# Autodesk Inventor assembly: SAR320
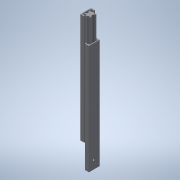
[picture p0: Inventor's stored thumbnail of the model, 180x180]
Saved by Autodesk Inventor 2020 (Build 240168000, 168)
## iProperties
Created: 2020-01-12
Part Number: SAR320
Catalog Web Link: www.cadenas.de
Description: SAR3-Slide Rails - Aluminum Alloy - Three-Step Slide Rails
Vendor: MISUMI
Document SubType Name: Assembly
Designer: psadmin
Manufacturer: MISUMI
Category: PARTsolutions
Company: MISUMI
PSOL_IDENT_0: {$CADENAS_DATA\23d-libs\misumi\metric\07_slide_rails\sar3_asmtab.prj},168 {VTYP=3D},{STYP=ASSTAB},{N
PSOL_IDENT_1: B=SAR320},{LINA=SAR320},{NN=SAR3},{DATE=09.09.2019 15:26:52},{GEOMDATE=01.03.2017 00:48:28},{VERSION=
PSOL_IDENT_2: },{LINEID=10},{WBVAR=NO},{WBNUMERIC=NO}  {NB=SAR320},{LINA=SAR320},{KT=DUMMY},{PN=SAR320},{TP=SAR3},
PSOL_IDENT_3: {TYPE=SAR3},{MAT1=Aluminum Alloy},{ST1=Clear Anodizing},{MAT2=Aluminum Alloy},{ST2=Clear Anodizing},
PSOL_IDENT_4: {MAT3=Steel},{NO=20},{RL=200},{TD=223},{A=85},{B=170},{C=85},{D=170},{RLO=147},{PPATH=sar3_series\\s
PSOL_IDENT_5: ar3_templ.prj}
NN: SAR3
NT: Slide Rails - Aluminum Alloy - Three-Step Slide Rails
NB: SAR320
NBSYN: $PN.
LINA: SAR320
PN: SAR320
TP: SAR3
MAT1: Aluminum Alloy
ST1: Clear Anodizing
MAT2: Aluminum Alloy
ST2: Clear Anodizing
MAT3: Steel
NO: 20
RL: 200
TD: 223
A: 85
B: 170
C: 85
D: 170
RLO: 147
SUPPLIER: MISUMI
ARTICLENO: SAR320
BOMINFO: SAR320
CREATOR: CADENAS GmbH
Title: SAR320
Author: Cadenas PARTsolutions
Comments: Slide Rails - Aluminum Alloy - Three-Step Slide Rails
## Documents named in this file (4)
- C:\Users\tdmp4\OneDrive\Documents\GitHub\CAD-2020\Misumi\SAR320.iam
- C:\Users\tdmp4\Downloads\SAR320_Autodesk_Inventor_2018_20200112\AIS2018\SAR320-20_r.ipt
- C:\Users\tdmp4\Downloads\SAR320_Autodesk_Inventor_2018_20200112\AIS2018\SAR320-20_b.ipt
- C:\Users\tdmp4\Downloads\SAR320_Autodesk_Inventor_2018_20200112\AIS2018\SAR3_ba.ipt
## Components (71 placed, 3 different names)
1. SAR320-20_r:1 — to_body_Z@1 <-> to_rail_Z@2, to_body_YZ@1 <-> to_rail_YZ@2, to_body2_Z@1 <-> to_rail_Z@3, to_body2_YZ@1 <-> to_rail_YZ@3, to_ball1_1_XY@1 <-> to_rail_XY@4, to_ball1_1_Z@1 <-> to_rail_Z@4, to_ball1_1_YZ@1 <-> to_rail_YZ@4, to_ball1_2_XY@1 <-> to_rail_XY@5, to_ball1_2_Z@1 <-> to_rail_Z@5, to_ball1_2_YZ@1 <-> to_rail_YZ@5, to_ball1_3_XY@1 <-> to_rail_XY@6, to_ball1_3_Z@1 <-> to_rail_Z@6, to_ball1_3_YZ@1 <-> to_rail_YZ@6, to_ball1_4_XY@1 <-> to_rail_XY@7, to_ball1_4_Z@1 <-> to_rail_Z@7, to_ball1_4_YZ@1 <-> to_rail_YZ@7, to_ball1_5_XY@1 <-> to_rail_XY@8, to_ball1_5_Z@1 <-> to_rail_Z@8, to_ball1_5_YZ@1 <-> to_rail_YZ@8, to_ball1_6_XY@1 <-> to_rail_XY@9, to_ball1_6_Z@1 <-> to_rail_Z@9, to_ball1_6_YZ@1 <-> to_rail_YZ@9, to_ball1_7_XY@1 <-> to_rail_XY@10, to_ball1_7_Z@1 <-> to_rail_Z@10, to_ball1_7_YZ@1 <-> to_rail_YZ@10, to_ball1_8_XY@1 <-> to_rail_XY@11, to_ball1_8_Z@1 <-> to_rail_Z@11, to_ball1_8_YZ@1 <-> to_rail_YZ@11, to_ball1_9_XY@1 <-> to_rail_XY@12, to_ball1_9_Z@1 <-> to_rail_Z@12, to_ball1_9_YZ@1 <-> to_rail_YZ@12, to_ball1_10_XY@1 <-> to_rail_XY@13, to_ball1_10_Z@1 <-> to_rail_Z@13, to_ball1_10_YZ@1 <-> to_rail_YZ@13, to_ball1_11_XY@1 <-> to_rail_XY@14, to_ball1_11_Z@1 <-> to_rail_Z@14, to_ball1_11_YZ@1 <-> to_rail_YZ@14, to_ball1_12_XY@1 <-> to_rail_XY@15, to_ball1_12_Z@1 <-> to_rail_Z@15, to_ball1_12_YZ@1 <-> to_rail_YZ@15, to_ball1_13_XY@1 <-> to_rail_XY@16, to_ball1_13_Z@1 <-> to_rail_Z@16, to_ball1_13_YZ@1 <-> to_rail_YZ@16, to_ball1_14_XY@1 <-> to_rail_XY@17, to_ball1_14_Z@1 <-> to_rail_Z@17, to_ball1_14_YZ@1 <-> to_rail_YZ@17, to_ball1_15_XY@1 <-> to_rail_XY@18, to_ball1_15_Z@1 <-> to_rail_Z@18, to_ball1_15_YZ@1 <-> to_rail_YZ@18, to_ball1_16_XY@1 <-> to_rail_XY@19, to_ball1_16_Z@1 <-> to_rail_Z@19, to_ball1_16_YZ@1 <-> to_rail_YZ@19, to_ball1_17_XY@1 <-> to_rail_XY@20, to_ball1_17_Z@1 <-> to_rail_Z@20, to_ball1_17_YZ@1 <-> to_rail_YZ@20, to_ball2_1_XY@1 <-> to_rail_XY@21, to_ball2_1_Z@1 <-> to_rail_Z@21, to_ball2_1_YZ@1 <-> to_rail_YZ@21, to_ball2_2_XY@1 <-> to_rail_XY@22, to_ball2_2_Z@1 <-> to_rail_Z@22, to_ball2_2_YZ@1 <-> to_rail_YZ@22, to_ball2_3_XY@1 <-> to_rail_XY@23, to_ball2_3_Z@1 <-> to_rail_Z@23, to_ball2_3_YZ@1 <-> to_rail_YZ@23, to_ball2_4_XY@1 <-> to_rail_XY@24, to_ball2_4_Z@1 <-> to_rail_Z@24, to_ball2_4_YZ@1 <-> to_rail_YZ@24, to_ball2_5_XY@1 <-> to_rail_XY@25, to_ball2_5_Z@1 <-> to_rail_Z@25, to_ball2_5_YZ@1 <-> to_rail_YZ@25, to_ball2_6_XY@1 <-> to_rail_XY@26, to_ball2_6_Z@1 <-> to_rail_Z@26, to_ball2_6_YZ@1 <-> to_rail_YZ@26, to_ball2_7_XY@1 <-> to_rail_XY@27, to_ball2_7_Z@1 <-> to_rail_Z@27, to_ball2_7_YZ@1 <-> to_rail_YZ@27, to_ball2_8_XY@1 <-> to_rail_XY@28, to_ball2_8_Z@1 <-> to_rail_Z@28, to_ball2_8_YZ@1 <-> to_rail_YZ@28, to_ball2_9_XY@1 <-> to_rail_XY@29, to_ball2_9_Z@1 <-> to_rail_Z@29, to_ball2_9_YZ@1 <-> to_rail_YZ@29, to_ball2_10_XY@1 <-> to_rail_XY@30, to_ball2_10_Z@1 <-> to_rail_Z@30, to_ball2_10_YZ@1 <-> to_rail_YZ@30, to_ball2_11_XY@1 <-> to_rail_XY@31, to_ball2_11_Z@1 <-> to_rail_Z@31, to_ball2_11_YZ@1 <-> to_rail_YZ@31, to_ball2_12_XY@1 <-> to_rail_XY@32, to_ball2_12_Z@1 <-> to_rail_Z@32, to_ball2_12_YZ@1 <-> to_rail_YZ@32, to_ball2_13_XY@1 <-> to_rail_XY@33, to_ball2_13_Z@1 <-> to_rail_Z@33, to_ball2_13_YZ@1 <-> to_rail_YZ@33, to_ball2_14_XY@1 <-> to_rail_XY@34, to_ball2_14_Z@1 <-> to_rail_Z@34, to_ball2_14_YZ@1 <-> to_rail_YZ@34, to_ball2_15_XY@1 <-> to_rail_XY@35, to_ball2_15_Z@1 <-> to_rail_Z@35, to_ball2_15_YZ@1 <-> to_rail_YZ@35, to_ball2_16_XY@1 <-> to_rail_XY@36, to_ball2_16_Z@1 <-> to_rail_Z@36, to_ball2_16_YZ@1 <-> to_rail_YZ@36, to_ball2_17_XY@1 <-> to_rail_XY@37, to_ball2_17_Z@1 <-> to_rail_Z@37, to_ball2_17_YZ@1 <-> to_rail_YZ@37, to_ball3_1_XY@1 <-> to_rail_XY@38, to_ball3_1_Z@1 <-> to_rail_Z@38, to_ball3_1_YZ@1 <-> to_rail_YZ@38, to_ball3_2_XY@1 <-> to_rail_XY@39, to_ball3_2_Z@1 <-> to_rail_Z@39, to_ball3_2_YZ@1 <-> to_rail_YZ@39, to_ball3_3_XY@1 <-> to_rail_XY@40, to_ball3_3_Z@1 <-> to_rail_Z@40, to_ball3_3_YZ@1 <-> to_rail_YZ@40, to_ball3_4_XY@1 <-> to_rail_XY@41, to_ball3_4_Z@1 <-> to_rail_Z@41, to_ball3_4_YZ@1 <-> to_rail_YZ@41, to_ball3_5_XY@1 <-> to_rail_XY@42, to_ball3_5_Z@1 <-> to_rail_Z@42, to_ball3_5_YZ@1 <-> to_rail_YZ@42, to_ball3_6_XY@1 <-> to_rail_XY@43, to_ball3_6_Z@1 <-> to_rail_Z@43, to_ball3_6_YZ@1 <-> to_rail_YZ@43, to_ball3_7_XY@1 <-> to_rail_XY@44, to_ball3_7_Z@1 <-> to_rail_Z@44, to_ball3_7_YZ@1 <-> to_rail_YZ@44, to_ball3_8_XY@1 <-> to_rail_XY@45, to_ball3_8_Z@1 <-> to_rail_Z@45, to_ball3_8_YZ@1 <-> to_rail_YZ@45, to_ball3_9_XY@1 <-> to_rail_XY@46, to_ball3_9_Z@1 <-> to_rail_Z@46, to_ball3_9_YZ@1 <-> to_rail_YZ@46, to_ball3_10_XY@1 <-> to_rail_XY@47, to_ball3_10_Z@1 <-> to_rail_Z@47, to_ball3_10_YZ@1 <-> to_rail_YZ@47, to_ball3_11_XY@1 <-> to_rail_XY@48, to_ball3_11_Z@1 <-> to_rail_Z@48, to_ball3_11_YZ@1 <-> to_rail_YZ@48, to_ball3_12_XY@1 <-> to_rail_XY@49, to_ball3_12_Z@1 <-> to_rail_Z@49, to_ball3_12_YZ@1 <-> to_rail_YZ@49, to_ball3_13_XY@1 <-> to_rail_XY@50, to_ball3_13_Z@1 <-> to_rail_Z@50, to_ball3_13_YZ@1 <-> to_rail_YZ@50, to_ball3_14_XY@1 <-> to_rail_XY@51, to_ball3_14_Z@1 <-> to_rail_Z@51, to_ball3_14_YZ@1 <-> to_rail_YZ@51, to_ball3_15_XY@1 <-> to_rail_XY@52, to_ball3_15_Z@1 <-> to_rail_Z@52, to_ball3_15_YZ@1 <-> to_rail_YZ@52, to_ball3_16_XY@1 <-> to_rail_XY@53, to_ball3_16_Z@1 <-> to_rail_Z@53, to_ball3_16_YZ@1 <-> to_rail_YZ@53, to_ball3_17_XY@1 <-> to_rail_XY@54, to_ball3_17_Z@1 <-> to_rail_Z@54, to_ball3_17_YZ@1 <-> to_rail_YZ@54, to_ball4_1_XY@1 <-> to_rail_XY@55, to_ball4_1_Z@1 <-> to_rail_Z@55, to_ball4_1_YZ@1 <-> to_rail_YZ@55, to_ball4_2_XY@1 <-> to_rail_XY@56, to_ball4_2_Z@1 <-> to_rail_Z@56, to_ball4_2_YZ@1 <-> to_rail_YZ@56, to_ball4_3_XY@1 <-> to_rail_XY@57, to_ball4_3_Z@1 <-> to_rail_Z@57, to_ball4_3_YZ@1 <-> to_rail_YZ@57, to_ball4_4_XY@1 <-> to_rail_XY@58, to_ball4_4_Z@1 <-> to_rail_Z@58, to_ball4_4_YZ@1 <-> to_rail_YZ@58, to_ball4_5_XY@1 <-> to_rail_XY@59, to_ball4_5_Z@1 <-> to_rail_Z@59, to_ball4_5_YZ@1 <-> to_rail_YZ@59, to_ball4_6_XY@1 <-> to_rail_XY@60, to_ball4_6_Z@1 <-> to_rail_Z@60, to_ball4_6_YZ@1 <-> to_rail_YZ@60, to_ball4_7_XY@1 <-> to_rail_XY@61, to_ball4_7_Z@1 <-> to_rail_Z@61, to_ball4_7_YZ@1 <-> to_rail_YZ@61, to_ball4_8_XY@1 <-> to_rail_XY@62, to_ball4_8_Z@1 <-> to_rail_Z@62, to_ball4_8_YZ@1 <-> to_rail_YZ@62, to_ball4_9_XY@1 <-> to_rail_XY@63, to_ball4_9_Z@1 <-> to_rail_Z@63, to_ball4_9_YZ@1 <-> to_rail_YZ@63, to_ball4_10_XY@1 <-> to_rail_XY@64, to_ball4_10_Z@1 <-> to_rail_Z@64, to_ball4_10_YZ@1 <-> to_rail_YZ@64, to_ball4_11_XY@1 <-> to_rail_XY@65, to_ball4_11_Z@1 <-> to_rail_Z@65, to_ball4_11_YZ@1 <-> to_rail_YZ@65, to_ball4_12_XY@1 <-> to_rail_XY@66, to_ball4_12_Z@1 <-> to_rail_Z@66, to_ball4_12_YZ@1 <-> to_rail_YZ@66, to_ball4_13_XY@1 <-> to_rail_XY@67, to_ball4_13_Z@1 <-> to_rail_Z@67, to_ball4_13_YZ@1 <-> to_rail_YZ@67, to_ball4_14_XY@1 <-> to_rail_XY@68, to_ball4_14_Z@1 <-> to_rail_Z@68, to_ball4_14_YZ@1 <-> to_rail_YZ@68, to_ball4_15_XY@1 <-> to_rail_XY@69, to_ball4_15_Z@1 <-> to_rail_Z@69, to_ball4_15_YZ@1 <-> to_rail_YZ@69, to_ball4_16_XY@1 <-> to_rail_XY@70, to_ball4_16_Z@1 <-> to_rail_Z@70, to_ball4_16_YZ@1 <-> to_rail_YZ@70, to_ball4_17_XY@1 <-> to_rail_XY@71, to_ball4_17_Z@1 <-> to_rail_Z@71, to_ball4_17_YZ@1 <-> to_rail_YZ@71
2. SAR320-20_b:1 — to_body_Z@1 <-> to_rail_Z@2, to_body_YZ@1 <-> to_rail_YZ@2
3. SAR320-20_b:2 — to_body2_Z@1 <-> to_rail_Z@3, to_body2_YZ@1 <-> to_rail_YZ@3
4. SAR3_ba:1 — to_ball1_1_XY@1 <-> to_rail_XY@4, to_ball1_1_Z@1 <-> to_rail_Z@4, to_ball1_1_YZ@1 <-> to_rail_YZ@4
5. SAR3_ba:2 — to_ball1_2_XY@1 <-> to_rail_XY@5, to_ball1_2_Z@1 <-> to_rail_Z@5, to_ball1_2_YZ@1 <-> to_rail_YZ@5
6. SAR3_ba:3 — to_ball1_3_XY@1 <-> to_rail_XY@6, to_ball1_3_Z@1 <-> to_rail_Z@6, to_ball1_3_YZ@1 <-> to_rail_YZ@6
7. SAR3_ba:4 — to_ball1_4_XY@1 <-> to_rail_XY@7, to_ball1_4_Z@1 <-> to_rail_Z@7, to_ball1_4_YZ@1 <-> to_rail_YZ@7
8. SAR3_ba:5 — to_ball1_5_XY@1 <-> to_rail_XY@8, to_ball1_5_Z@1 <-> to_rail_Z@8, to_ball1_5_YZ@1 <-> to_rail_YZ@8
9. SAR3_ba:6 — to_ball1_6_XY@1 <-> to_rail_XY@9, to_ball1_6_Z@1 <-> to_rail_Z@9, to_ball1_6_YZ@1 <-> to_rail_YZ@9
10. SAR3_ba:7 — to_ball1_7_XY@1 <-> to_rail_XY@10, to_ball1_7_Z@1 <-> to_rail_Z@10, to_ball1_7_YZ@1 <-> to_rail_YZ@10
11. SAR3_ba:8 — to_ball1_8_XY@1 <-> to_rail_XY@11, to_ball1_8_Z@1 <-> to_rail_Z@11, to_ball1_8_YZ@1 <-> to_rail_YZ@11
12. SAR3_ba:9 — to_ball1_9_XY@1 <-> to_rail_XY@12, to_ball1_9_Z@1 <-> to_rail_Z@12, to_ball1_9_YZ@1 <-> to_rail_YZ@12
13. SAR3_ba:10 — to_ball1_10_XY@1 <-> to_rail_XY@13, to_ball1_10_Z@1 <-> to_rail_Z@13, to_ball1_10_YZ@1 <-> to_rail_YZ@13
14. SAR3_ba:11 — to_ball1_11_XY@1 <-> to_rail_XY@14, to_ball1_11_Z@1 <-> to_rail_Z@14, to_ball1_11_YZ@1 <-> to_rail_YZ@14
15. SAR3_ba:12 — to_ball1_12_XY@1 <-> to_rail_XY@15, to_ball1_12_Z@1 <-> to_rail_Z@15, to_ball1_12_YZ@1 <-> to_rail_YZ@15
16. SAR3_ba:13 — to_ball1_13_XY@1 <-> to_rail_XY@16, to_ball1_13_Z@1 <-> to_rail_Z@16, to_ball1_13_YZ@1 <-> to_rail_YZ@16
17. SAR3_ba:14 — to_ball1_14_XY@1 <-> to_rail_XY@17, to_ball1_14_Z@1 <-> to_rail_Z@17, to_ball1_14_YZ@1 <-> to_rail_YZ@17
18. SAR3_ba:15 — to_ball1_15_XY@1 <-> to_rail_XY@18, to_ball1_15_Z@1 <-> to_rail_Z@18, to_ball1_15_YZ@1 <-> to_rail_YZ@18
19. SAR3_ba:16 — to_ball1_16_XY@1 <-> to_rail_XY@19, to_ball1_16_Z@1 <-> to_rail_Z@19, to_ball1_16_YZ@1 <-> to_rail_YZ@19
20. SAR3_ba:17 — to_ball1_17_XY@1 <-> to_rail_XY@20, to_ball1_17_Z@1 <-> to_rail_Z@20, to_ball1_17_YZ@1 <-> to_rail_YZ@20
21. SAR3_ba:18 — to_ball2_1_XY@1 <-> to_rail_XY@21, to_ball2_1_Z@1 <-> to_rail_Z@21, to_ball2_1_YZ@1 <-> to_rail_YZ@21
22. SAR3_ba:19 — to_ball2_2_XY@1 <-> to_rail_XY@22, to_ball2_2_Z@1 <-> to_rail_Z@22, to_ball2_2_YZ@1 <-> to_rail_YZ@22
23. SAR3_ba:20 — to_ball2_3_XY@1 <-> to_rail_XY@23, to_ball2_3_Z@1 <-> to_rail_Z@23, to_ball2_3_YZ@1 <-> to_rail_YZ@23
24. SAR3_ba:21 — to_ball2_4_XY@1 <-> to_rail_XY@24, to_ball2_4_Z@1 <-> to_rail_Z@24, to_ball2_4_YZ@1 <-> to_rail_YZ@24
25. SAR3_ba:22 — to_ball2_5_XY@1 <-> to_rail_XY@25, to_ball2_5_Z@1 <-> to_rail_Z@25, to_ball2_5_YZ@1 <-> to_rail_YZ@25
26. SAR3_ba:23 — to_ball2_6_XY@1 <-> to_rail_XY@26, to_ball2_6_Z@1 <-> to_rail_Z@26, to_ball2_6_YZ@1 <-> to_rail_YZ@26
27. SAR3_ba:24 — to_ball2_7_XY@1 <-> to_rail_XY@27, to_ball2_7_Z@1 <-> to_rail_Z@27, to_ball2_7_YZ@1 <-> to_rail_YZ@27
28. SAR3_ba:25 — to_ball2_8_XY@1 <-> to_rail_XY@28, to_ball2_8_Z@1 <-> to_rail_Z@28, to_ball2_8_YZ@1 <-> to_rail_YZ@28
29. SAR3_ba:26 — to_ball2_9_XY@1 <-> to_rail_XY@29, to_ball2_9_Z@1 <-> to_rail_Z@29, to_ball2_9_YZ@1 <-> to_rail_YZ@29
30. SAR3_ba:27 — to_ball2_10_XY@1 <-> to_rail_XY@30, to_ball2_10_Z@1 <-> to_rail_Z@30, to_ball2_10_YZ@1 <-> to_rail_YZ@30
31. SAR3_ba:28 — to_ball2_11_XY@1 <-> to_rail_XY@31, to_ball2_11_Z@1 <-> to_rail_Z@31, to_ball2_11_YZ@1 <-> to_rail_YZ@31
32. SAR3_ba:29 — to_ball2_12_XY@1 <-> to_rail_XY@32, to_ball2_12_Z@1 <-> to_rail_Z@32, to_ball2_12_YZ@1 <-> to_rail_YZ@32
33. SAR3_ba:30 — to_ball2_13_XY@1 <-> to_rail_XY@33, to_ball2_13_Z@1 <-> to_rail_Z@33, to_ball2_13_YZ@1 <-> to_rail_YZ@33
34. SAR3_ba:31 — to_ball2_14_XY@1 <-> to_rail_XY@34, to_ball2_14_Z@1 <-> to_rail_Z@34, to_ball2_14_YZ@1 <-> to_rail_YZ@34
35. SAR3_ba:32 — to_ball2_15_XY@1 <-> to_rail_XY@35, to_ball2_15_Z@1 <-> to_rail_Z@35, to_ball2_15_YZ@1 <-> to_rail_YZ@35
36. SAR3_ba:33 — to_ball2_16_XY@1 <-> to_rail_XY@36, to_ball2_16_Z@1 <-> to_rail_Z@36, to_ball2_16_YZ@1 <-> to_rail_YZ@36
37. SAR3_ba:34 — to_ball2_17_XY@1 <-> to_rail_XY@37, to_ball2_17_Z@1 <-> to_rail_Z@37, to_ball2_17_YZ@1 <-> to_rail_YZ@37
38. SAR3_ba:35 — to_ball3_1_XY@1 <-> to_rail_XY@38, to_ball3_1_Z@1 <-> to_rail_Z@38, to_ball3_1_YZ@1 <-> to_rail_YZ@38
39. SAR3_ba:36 — to_ball3_2_XY@1 <-> to_rail_XY@39, to_ball3_2_Z@1 <-> to_rail_Z@39, to_ball3_2_YZ@1 <-> to_rail_YZ@39
40. SAR3_ba:37 — to_ball3_3_XY@1 <-> to_rail_XY@40, to_ball3_3_Z@1 <-> to_rail_Z@40, to_ball3_3_YZ@1 <-> to_rail_YZ@40
41. SAR3_ba:38 — to_ball3_4_XY@1 <-> to_rail_XY@41, to_ball3_4_Z@1 <-> to_rail_Z@41, to_ball3_4_YZ@1 <-> to_rail_YZ@41
42. SAR3_ba:39 — to_ball3_5_XY@1 <-> to_rail_XY@42, to_ball3_5_Z@1 <-> to_rail_Z@42, to_ball3_5_YZ@1 <-> to_rail_YZ@42
43. SAR3_ba:40 — to_ball3_6_XY@1 <-> to_rail_XY@43, to_ball3_6_Z@1 <-> to_rail_Z@43, to_ball3_6_YZ@1 <-> to_rail_YZ@43
44. SAR3_ba:41 — to_ball3_7_XY@1 <-> to_rail_XY@44, to_ball3_7_Z@1 <-> to_rail_Z@44, to_ball3_7_YZ@1 <-> to_rail_YZ@44
45. SAR3_ba:42 — to_ball3_8_XY@1 <-> to_rail_XY@45, to_ball3_8_Z@1 <-> to_rail_Z@45, to_ball3_8_YZ@1 <-> to_rail_YZ@45
46. SAR3_ba:43 — to_ball3_9_XY@1 <-> to_rail_XY@46, to_ball3_9_Z@1 <-> to_rail_Z@46, to_ball3_9_YZ@1 <-> to_rail_YZ@46
47. SAR3_ba:44 — to_ball3_10_XY@1 <-> to_rail_XY@47, to_ball3_10_Z@1 <-> to_rail_Z@47, to_ball3_10_YZ@1 <-> to_rail_YZ@47
48. SAR3_ba:45 — to_ball3_11_XY@1 <-> to_rail_XY@48, to_ball3_11_Z@1 <-> to_rail_Z@48, to_ball3_11_YZ@1 <-> to_rail_YZ@48
49. SAR3_ba:46 — to_ball3_12_XY@1 <-> to_rail_XY@49, to_ball3_12_Z@1 <-> to_rail_Z@49, to_ball3_12_YZ@1 <-> to_rail_YZ@49
50. SAR3_ba:47 — to_ball3_13_XY@1 <-> to_rail_XY@50, to_ball3_13_Z@1 <-> to_rail_Z@50, to_ball3_13_YZ@1 <-> to_rail_YZ@50
51. SAR3_ba:48 — to_ball3_14_XY@1 <-> to_rail_XY@51, to_ball3_14_Z@1 <-> to_rail_Z@51, to_ball3_14_YZ@1 <-> to_rail_YZ@51
52. SAR3_ba:49 — to_ball3_15_XY@1 <-> to_rail_XY@52, to_ball3_15_Z@1 <-> to_rail_Z@52, to_ball3_15_YZ@1 <-> to_rail_YZ@52
53. SAR3_ba:50 — to_ball3_16_XY@1 <-> to_rail_XY@53, to_ball3_16_Z@1 <-> to_rail_Z@53, to_ball3_16_YZ@1 <-> to_rail_YZ@53
54. SAR3_ba:51 — to_ball3_17_XY@1 <-> to_rail_XY@54, to_ball3_17_Z@1 <-> to_rail_Z@54, to_ball3_17_YZ@1 <-> to_rail_YZ@54
55. SAR3_ba:52 — to_ball4_1_XY@1 <-> to_rail_XY@55, to_ball4_1_Z@1 <-> to_rail_Z@55, to_ball4_1_YZ@1 <-> to_rail_YZ@55
56. SAR3_ba:53 — to_ball4_2_XY@1 <-> to_rail_XY@56, to_ball4_2_Z@1 <-> to_rail_Z@56, to_ball4_2_YZ@1 <-> to_rail_YZ@56
57. SAR3_ba:54 — to_ball4_3_XY@1 <-> to_rail_XY@57, to_ball4_3_Z@1 <-> to_rail_Z@57, to_ball4_3_YZ@1 <-> to_rail_YZ@57
58. SAR3_ba:55 — to_ball4_4_XY@1 <-> to_rail_XY@58, to_ball4_4_Z@1 <-> to_rail_Z@58, to_ball4_4_YZ@1 <-> to_rail_YZ@58
59. SAR3_ba:56 — to_ball4_5_XY@1 <-> to_rail_XY@59, to_ball4_5_Z@1 <-> to_rail_Z@59, to_ball4_5_YZ@1 <-> to_rail_YZ@59
60. SAR3_ba:57 — to_ball4_6_XY@1 <-> to_rail_XY@60, to_ball4_6_Z@1 <-> to_rail_Z@60, to_ball4_6_YZ@1 <-> to_rail_YZ@60
61. SAR3_ba:58 — to_ball4_7_XY@1 <-> to_rail_XY@61, to_ball4_7_Z@1 <-> to_rail_Z@61, to_ball4_7_YZ@1 <-> to_rail_YZ@61
62. SAR3_ba:59 — to_ball4_8_XY@1 <-> to_rail_XY@62, to_ball4_8_Z@1 <-> to_rail_Z@62, to_ball4_8_YZ@1 <-> to_rail_YZ@62
63. SAR3_ba:60 — to_ball4_9_XY@1 <-> to_rail_XY@63, to_ball4_9_Z@1 <-> to_rail_Z@63, to_ball4_9_YZ@1 <-> to_rail_YZ@63
64. SAR3_ba:61 — to_ball4_10_XY@1 <-> to_rail_XY@64, to_ball4_10_Z@1 <-> to_rail_Z@64, to_ball4_10_YZ@1 <-> to_rail_YZ@64
65. SAR3_ba:62 — to_ball4_11_XY@1 <-> to_rail_XY@65, to_ball4_11_Z@1 <-> to_rail_Z@65, to_ball4_11_YZ@1 <-> to_rail_YZ@65
66. SAR3_ba:63 — to_ball4_12_XY@1 <-> to_rail_XY@66, to_ball4_12_Z@1 <-> to_rail_Z@66, to_ball4_12_YZ@1 <-> to_rail_YZ@66
67. SAR3_ba:64 — to_ball4_13_XY@1 <-> to_rail_XY@67, to_ball4_13_Z@1 <-> to_rail_Z@67, to_ball4_13_YZ@1 <-> to_rail_YZ@67
68. SAR3_ba:65 — to_ball4_14_XY@1 <-> to_rail_XY@68, to_ball4_14_Z@1 <-> to_rail_Z@68, to_ball4_14_YZ@1 <-> to_rail_YZ@68
69. SAR3_ba:66 — to_ball4_15_XY@1 <-> to_rail_XY@69, to_ball4_15_Z@1 <-> to_rail_Z@69, to_ball4_15_YZ@1 <-> to_rail_YZ@69
70. SAR3_ba:67 — to_ball4_16_XY@1 <-> to_rail_XY@70, to_ball4_16_Z@1 <-> to_rail_Z@70, to_ball4_16_YZ@1 <-> to_rail_YZ@70
71. SAR3_ba:68 — to_ball4_17_XY@1 <-> to_rail_XY@71, to_ball4_17_Z@1 <-> to_rail_Z@71, to_ball4_17_YZ@1 <-> to_rail_YZ@71
## Relationships (208: Mate 138, Angle 70)
- to_body_Z@1 <-> to_rail_Z@2 [Mate]: SAR320-20_r:1 ↔ SAR320-20_b:1
- to_body_YZ@1 <-> to_rail_YZ@2 [Angle] (0 deg): SAR320-20_r:1 ↔ SAR320-20_b:1
- to_body2_Z@1 <-> to_rail_Z@3 [Mate]: SAR320-20_r:1 ↔ SAR320-20_b:2
- to_body2_YZ@1 <-> to_rail_YZ@3 [Angle] (180 deg): SAR320-20_r:1 ↔ SAR320-20_b:2
- to_ball1_1_XY@1 <-> to_rail_XY@4 [Mate]: SAR320-20_r:1 ↔ SAR3_ba:1
- to_ball1_1_Z@1 <-> to_rail_Z@4 [Mate]: SAR320-20_r:1 ↔ SAR3_ba:1
- to_ball1_1_YZ@1 <-> to_rail_YZ@4 [Angle] (0 deg): SAR320-20_r:1 ↔ SAR3_ba:1
- to_ball1_2_XY@1 <-> to_rail_XY@5 [Mate]: SAR320-20_r:1 ↔ SAR3_ba:2
- to_ball1_2_Z@1 <-> to_rail_Z@5 [Mate]: SAR320-20_r:1 ↔ SAR3_ba:2
- to_ball1_2_YZ@1 <-> to_rail_YZ@5 [Angle] (0 deg): SAR320-20_r:1 ↔ SAR3_ba:2
- to_ball1_3_XY@1 <-> to_rail_XY@6 [Mate]: SAR320-20_r:1 ↔ SAR3_ba:3
- to_ball1_3_Z@1 <-> to_rail_Z@6 [Mate]: SAR320-20_r:1 ↔ SAR3_ba:3
- to_ball1_3_YZ@1 <-> to_rail_YZ@6 [Angle] (0 deg): SAR320-20_r:1 ↔ SAR3_ba:3
- to_ball1_4_XY@1 <-> to_rail_XY@7 [Mate]: SAR320-20_r:1 ↔ SAR3_ba:4
- to_ball1_4_Z@1 <-> to_rail_Z@7 [Mate]: SAR320-20_r:1 ↔ SAR3_ba:4
- to_ball1_4_YZ@1 <-> to_rail_YZ@7 [Angle] (0 deg): SAR320-20_r:1 ↔ SAR3_ba:4
- to_ball1_5_XY@1 <-> to_rail_XY@8 [Mate]: SAR320-20_r:1 ↔ SAR3_ba:5
- to_ball1_5_Z@1 <-> to_rail_Z@8 [Mate]: SAR320-20_r:1 ↔ SAR3_ba:5
- to_ball1_5_YZ@1 <-> to_rail_YZ@8 [Angle] (0 deg): SAR320-20_r:1 ↔ SAR3_ba:5
- to_ball1_6_XY@1 <-> to_rail_XY@9 [Mate]: SAR320-20_r:1 ↔ SAR3_ba:6
- to_ball1_6_Z@1 <-> to_rail_Z@9 [Mate]: SAR320-20_r:1 ↔ SAR3_ba:6
- to_ball1_6_YZ@1 <-> to_rail_YZ@9 [Angle] (0 deg): SAR320-20_r:1 ↔ SAR3_ba:6
- to_ball1_7_XY@1 <-> to_rail_XY@10 [Mate]: SAR320-20_r:1 ↔ SAR3_ba:7
- to_ball1_7_Z@1 <-> to_rail_Z@10 [Mate]: SAR320-20_r:1 ↔ SAR3_ba:7
- to_ball1_7_YZ@1 <-> to_rail_YZ@10 [Angle] (0 deg): SAR320-20_r:1 ↔ SAR3_ba:7
- to_ball1_8_XY@1 <-> to_rail_XY@11 [Mate]: SAR320-20_r:1 ↔ SAR3_ba:8
- to_ball1_8_Z@1 <-> to_rail_Z@11 [Mate]: SAR320-20_r:1 ↔ SAR3_ba:8
- to_ball1_8_YZ@1 <-> to_rail_YZ@11 [Angle] (0 deg): SAR320-20_r:1 ↔ SAR3_ba:8
- to_ball1_9_XY@1 <-> to_rail_XY@12 [Mate]: SAR320-20_r:1 ↔ SAR3_ba:9
- to_ball1_9_Z@1 <-> to_rail_Z@12 [Mate]: SAR320-20_r:1 ↔ SAR3_ba:9
- to_ball1_9_YZ@1 <-> to_rail_YZ@12 [Angle] (0 deg): SAR320-20_r:1 ↔ SAR3_ba:9
- to_ball1_10_XY@1 <-> to_rail_XY@13 [Mate]: SAR320-20_r:1 ↔ SAR3_ba:10
- to_ball1_10_Z@1 <-> to_rail_Z@13 [Mate]: SAR320-20_r:1 ↔ SAR3_ba:10
- to_ball1_10_YZ@1 <-> to_rail_YZ@13 [Angle] (0 deg): SAR320-20_r:1 ↔ SAR3_ba:10
- to_ball1_11_XY@1 <-> to_rail_XY@14 [Mate]: SAR320-20_r:1 ↔ SAR3_ba:11
- to_ball1_11_Z@1 <-> to_rail_Z@14 [Mate]: SAR320-20_r:1 ↔ SAR3_ba:11
- to_ball1_11_YZ@1 <-> to_rail_YZ@14 [Angle] (0 deg): SAR320-20_r:1 ↔ SAR3_ba:11
- to_ball1_12_XY@1 <-> to_rail_XY@15 [Mate]: SAR320-20_r:1 ↔ SAR3_ba:12
- to_ball1_12_Z@1 <-> to_rail_Z@15 [Mate]: SAR320-20_r:1 ↔ SAR3_ba:12
- to_ball1_12_YZ@1 <-> to_rail_YZ@15 [Angle] (0 deg): SAR320-20_r:1 ↔ SAR3_ba:12
- to_ball1_13_XY@1 <-> to_rail_XY@16 [Mate]: SAR320-20_r:1 ↔ SAR3_ba:13
- to_ball1_13_Z@1 <-> to_rail_Z@16 [Mate]: SAR320-20_r:1 ↔ SAR3_ba:13
- to_ball1_13_YZ@1 <-> to_rail_YZ@16 [Angle] (0 deg): SAR320-20_r:1 ↔ SAR3_ba:13
- to_ball1_14_XY@1 <-> to_rail_XY@17 [Mate]: SAR320-20_r:1 ↔ SAR3_ba:14
- to_ball1_14_Z@1 <-> to_rail_Z@17 [Mate]: SAR320-20_r:1 ↔ SAR3_ba:14
- to_ball1_14_YZ@1 <-> to_rail_YZ@17 [Angle] (0 deg): SAR320-20_r:1 ↔ SAR3_ba:14
- to_ball1_15_XY@1 <-> to_rail_XY@18 [Mate]: SAR320-20_r:1 ↔ SAR3_ba:15
- to_ball1_15_Z@1 <-> to_rail_Z@18 [Mate]: SAR320-20_r:1 ↔ SAR3_ba:15
- to_ball1_15_YZ@1 <-> to_rail_YZ@18 [Angle] (0 deg): SAR320-20_r:1 ↔ SAR3_ba:15
- to_ball1_16_XY@1 <-> to_rail_XY@19 [Mate]: SAR320-20_r:1 ↔ SAR3_ba:16
- to_ball1_16_Z@1 <-> to_rail_Z@19 [Mate]: SAR320-20_r:1 ↔ SAR3_ba:16
- to_ball1_16_YZ@1 <-> to_rail_YZ@19 [Angle] (0 deg): SAR320-20_r:1 ↔ SAR3_ba:16
- to_ball1_17_XY@1 <-> to_rail_XY@20 [Mate]: SAR320-20_r:1 ↔ SAR3_ba:17
- to_ball1_17_Z@1 <-> to_rail_Z@20 [Mate]: SAR320-20_r:1 ↔ SAR3_ba:17
- to_ball1_17_YZ@1 <-> to_rail_YZ@20 [Angle] (0 deg): SAR320-20_r:1 ↔ SAR3_ba:17
- to_ball2_1_XY@1 <-> to_rail_XY@21 [Mate]: SAR320-20_r:1 ↔ SAR3_ba:18
- to_ball2_1_Z@1 <-> to_rail_Z@21 [Mate]: SAR320-20_r:1 ↔ SAR3_ba:18
- to_ball2_1_YZ@1 <-> to_rail_YZ@21 [Angle] (0 deg): SAR320-20_r:1 ↔ SAR3_ba:18
- to_ball2_2_XY@1 <-> to_rail_XY@22 [Mate]: SAR320-20_r:1 ↔ SAR3_ba:19
- to_ball2_2_Z@1 <-> to_rail_Z@22 [Mate]: SAR320-20_r:1 ↔ SAR3_ba:19
- to_ball2_2_YZ@1 <-> to_rail_YZ@22 [Angle] (0 deg): SAR320-20_r:1 ↔ SAR3_ba:19
- to_ball2_3_XY@1 <-> to_rail_XY@23 [Mate]: SAR320-20_r:1 ↔ SAR3_ba:20
- to_ball2_3_Z@1 <-> to_rail_Z@23 [Mate]: SAR320-20_r:1 ↔ SAR3_ba:20
- to_ball2_3_YZ@1 <-> to_rail_YZ@23 [Angle] (0 deg): SAR320-20_r:1 ↔ SAR3_ba:20
- to_ball2_4_XY@1 <-> to_rail_XY@24 [Mate]: SAR320-20_r:1 ↔ SAR3_ba:21
- to_ball2_4_Z@1 <-> to_rail_Z@24 [Mate]: SAR320-20_r:1 ↔ SAR3_ba:21
- to_ball2_4_YZ@1 <-> to_rail_YZ@24 [Angle] (0 deg): SAR320-20_r:1 ↔ SAR3_ba:21
- to_ball2_5_XY@1 <-> to_rail_XY@25 [Mate]: SAR320-20_r:1 ↔ SAR3_ba:22
- to_ball2_5_Z@1 <-> to_rail_Z@25 [Mate]: SAR320-20_r:1 ↔ SAR3_ba:22
- to_ball2_5_YZ@1 <-> to_rail_YZ@25 [Angle] (0 deg): SAR320-20_r:1 ↔ SAR3_ba:22
- to_ball2_6_XY@1 <-> to_rail_XY@26 [Mate]: SAR320-20_r:1 ↔ SAR3_ba:23
- to_ball2_6_Z@1 <-> to_rail_Z@26 [Mate]: SAR320-20_r:1 ↔ SAR3_ba:23
- to_ball2_6_YZ@1 <-> to_rail_YZ@26 [Angle] (0 deg): SAR320-20_r:1 ↔ SAR3_ba:23
- to_ball2_7_XY@1 <-> to_rail_XY@27 [Mate]: SAR320-20_r:1 ↔ SAR3_ba:24
- to_ball2_7_Z@1 <-> to_rail_Z@27 [Mate]: SAR320-20_r:1 ↔ SAR3_ba:24
- to_ball2_7_YZ@1 <-> to_rail_YZ@27 [Angle] (0 deg): SAR320-20_r:1 ↔ SAR3_ba:24
- to_ball2_8_XY@1 <-> to_rail_XY@28 [Mate]: SAR320-20_r:1 ↔ SAR3_ba:25
- to_ball2_8_Z@1 <-> to_rail_Z@28 [Mate]: SAR320-20_r:1 ↔ SAR3_ba:25
- to_ball2_8_YZ@1 <-> to_rail_YZ@28 [Angle] (0 deg): SAR320-20_r:1 ↔ SAR3_ba:25
- to_ball2_9_XY@1 <-> to_rail_XY@29 [Mate]: SAR320-20_r:1 ↔ SAR3_ba:26
- to_ball2_9_Z@1 <-> to_rail_Z@29 [Mate]: SAR320-20_r:1 ↔ SAR3_ba:26
- to_ball2_9_YZ@1 <-> to_rail_YZ@29 [Angle] (0 deg): SAR320-20_r:1 ↔ SAR3_ba:26
- to_ball2_10_XY@1 <-> to_rail_XY@30 [Mate]: SAR320-20_r:1 ↔ SAR3_ba:27
- to_ball2_10_Z@1 <-> to_rail_Z@30 [Mate]: SAR320-20_r:1 ↔ SAR3_ba:27
- to_ball2_10_YZ@1 <-> to_rail_YZ@30 [Angle] (0 deg): SAR320-20_r:1 ↔ SAR3_ba:27
- to_ball2_11_XY@1 <-> to_rail_XY@31 [Mate]: SAR320-20_r:1 ↔ SAR3_ba:28
- to_ball2_11_Z@1 <-> to_rail_Z@31 [Mate]: SAR320-20_r:1 ↔ SAR3_ba:28
- to_ball2_11_YZ@1 <-> to_rail_YZ@31 [Angle] (0 deg): SAR320-20_r:1 ↔ SAR3_ba:28
- to_ball2_12_XY@1 <-> to_rail_XY@32 [Mate]: SAR320-20_r:1 ↔ SAR3_ba:29
- to_ball2_12_Z@1 <-> to_rail_Z@32 [Mate]: SAR320-20_r:1 ↔ SAR3_ba:29
- to_ball2_12_YZ@1 <-> to_rail_YZ@32 [Angle] (0 deg): SAR320-20_r:1 ↔ SAR3_ba:29
- to_ball2_13_XY@1 <-> to_rail_XY@33 [Mate]: SAR320-20_r:1 ↔ SAR3_ba:30
- to_ball2_13_Z@1 <-> to_rail_Z@33 [Mate]: SAR320-20_r:1 ↔ SAR3_ba:30
- to_ball2_13_YZ@1 <-> to_rail_YZ@33 [Angle] (0 deg): SAR320-20_r:1 ↔ SAR3_ba:30
- to_ball2_14_XY@1 <-> to_rail_XY@34 [Mate]: SAR320-20_r:1 ↔ SAR3_ba:31
- to_ball2_14_Z@1 <-> to_rail_Z@34 [Mate]: SAR320-20_r:1 ↔ SAR3_ba:31
- to_ball2_14_YZ@1 <-> to_rail_YZ@34 [Angle] (0 deg): SAR320-20_r:1 ↔ SAR3_ba:31
- to_ball2_15_XY@1 <-> to_rail_XY@35 [Mate]: SAR320-20_r:1 ↔ SAR3_ba:32
- to_ball2_15_Z@1 <-> to_rail_Z@35 [Mate]: SAR320-20_r:1 ↔ SAR3_ba:32
- to_ball2_15_YZ@1 <-> to_rail_YZ@35 [Angle] (0 deg): SAR320-20_r:1 ↔ SAR3_ba:32
- to_ball2_16_XY@1 <-> to_rail_XY@36 [Mate]: SAR320-20_r:1 ↔ SAR3_ba:33
- to_ball2_16_Z@1 <-> to_rail_Z@36 [Mate]: SAR320-20_r:1 ↔ SAR3_ba:33
- to_ball2_16_YZ@1 <-> to_rail_YZ@36 [Angle] (0 deg): SAR320-20_r:1 ↔ SAR3_ba:33
- to_ball2_17_XY@1 <-> to_rail_XY@37 [Mate]: SAR320-20_r:1 ↔ SAR3_ba:34
- to_ball2_17_Z@1 <-> to_rail_Z@37 [Mate]: SAR320-20_r:1 ↔ SAR3_ba:34
- to_ball2_17_YZ@1 <-> to_rail_YZ@37 [Angle] (0 deg): SAR320-20_r:1 ↔ SAR3_ba:34
- to_ball3_1_XY@1 <-> to_rail_XY@38 [Mate]: SAR320-20_r:1 ↔ SAR3_ba:35
- to_ball3_1_Z@1 <-> to_rail_Z@38 [Mate]: SAR320-20_r:1 ↔ SAR3_ba:35
- to_ball3_1_YZ@1 <-> to_rail_YZ@38 [Angle] (0 deg): SAR320-20_r:1 ↔ SAR3_ba:35
- to_ball3_2_XY@1 <-> to_rail_XY@39 [Mate]: SAR320-20_r:1 ↔ SAR3_ba:36
- to_ball3_2_Z@1 <-> to_rail_Z@39 [Mate]: SAR320-20_r:1 ↔ SAR3_ba:36
- to_ball3_2_YZ@1 <-> to_rail_YZ@39 [Angle] (0 deg): SAR320-20_r:1 ↔ SAR3_ba:36
- to_ball3_3_XY@1 <-> to_rail_XY@40 [Mate]: SAR320-20_r:1 ↔ SAR3_ba:37
- to_ball3_3_Z@1 <-> to_rail_Z@40 [Mate]: SAR320-20_r:1 ↔ SAR3_ba:37
- to_ball3_3_YZ@1 <-> to_rail_YZ@40 [Angle] (0 deg): SAR320-20_r:1 ↔ SAR3_ba:37
- to_ball3_4_XY@1 <-> to_rail_XY@41 [Mate]: SAR320-20_r:1 ↔ SAR3_ba:38
- to_ball3_4_Z@1 <-> to_rail_Z@41 [Mate]: SAR320-20_r:1 ↔ SAR3_ba:38
- to_ball3_4_YZ@1 <-> to_rail_YZ@41 [Angle] (0 deg): SAR320-20_r:1 ↔ SAR3_ba:38
- to_ball3_5_XY@1 <-> to_rail_XY@42 [Mate]: SAR320-20_r:1 ↔ SAR3_ba:39
- to_ball3_5_Z@1 <-> to_rail_Z@42 [Mate]: SAR320-20_r:1 ↔ SAR3_ba:39
- to_ball3_5_YZ@1 <-> to_rail_YZ@42 [Angle] (0 deg): SAR320-20_r:1 ↔ SAR3_ba:39
- to_ball3_6_XY@1 <-> to_rail_XY@43 [Mate]: SAR320-20_r:1 ↔ SAR3_ba:40
- to_ball3_6_Z@1 <-> to_rail_Z@43 [Mate]: SAR320-20_r:1 ↔ SAR3_ba:40
- to_ball3_6_YZ@1 <-> to_rail_YZ@43 [Angle] (0 deg): SAR320-20_r:1 ↔ SAR3_ba:40
- to_ball3_7_XY@1 <-> to_rail_XY@44 [Mate]: SAR320-20_r:1 ↔ SAR3_ba:41
- to_ball3_7_Z@1 <-> to_rail_Z@44 [Mate]: SAR320-20_r:1 ↔ SAR3_ba:41
- to_ball3_7_YZ@1 <-> to_rail_YZ@44 [Angle] (0 deg): SAR320-20_r:1 ↔ SAR3_ba:41
- to_ball3_8_XY@1 <-> to_rail_XY@45 [Mate]: SAR320-20_r:1 ↔ SAR3_ba:42
- to_ball3_8_Z@1 <-> to_rail_Z@45 [Mate]: SAR320-20_r:1 ↔ SAR3_ba:42
- to_ball3_8_YZ@1 <-> to_rail_YZ@45 [Angle] (0 deg): SAR320-20_r:1 ↔ SAR3_ba:42
- to_ball3_9_XY@1 <-> to_rail_XY@46 [Mate]: SAR320-20_r:1 ↔ SAR3_ba:43
- to_ball3_9_Z@1 <-> to_rail_Z@46 [Mate]: SAR320-20_r:1 ↔ SAR3_ba:43
- to_ball3_9_YZ@1 <-> to_rail_YZ@46 [Angle] (0 deg): SAR320-20_r:1 ↔ SAR3_ba:43
- to_ball3_10_XY@1 <-> to_rail_XY@47 [Mate]: SAR320-20_r:1 ↔ SAR3_ba:44
- to_ball3_10_Z@1 <-> to_rail_Z@47 [Mate]: SAR320-20_r:1 ↔ SAR3_ba:44
- to_ball3_10_YZ@1 <-> to_rail_YZ@47 [Angle] (0 deg): SAR320-20_r:1 ↔ SAR3_ba:44
- to_ball3_11_XY@1 <-> to_rail_XY@48 [Mate]: SAR320-20_r:1 ↔ SAR3_ba:45
- to_ball3_11_Z@1 <-> to_rail_Z@48 [Mate]: SAR320-20_r:1 ↔ SAR3_ba:45
- to_ball3_11_YZ@1 <-> to_rail_YZ@48 [Angle] (0 deg): SAR320-20_r:1 ↔ SAR3_ba:45
- to_ball3_12_XY@1 <-> to_rail_XY@49 [Mate]: SAR320-20_r:1 ↔ SAR3_ba:46
- to_ball3_12_Z@1 <-> to_rail_Z@49 [Mate]: SAR320-20_r:1 ↔ SAR3_ba:46
- to_ball3_12_YZ@1 <-> to_rail_YZ@49 [Angle] (0 deg): SAR320-20_r:1 ↔ SAR3_ba:46
- to_ball3_13_XY@1 <-> to_rail_XY@50 [Mate]: SAR320-20_r:1 ↔ SAR3_ba:47
- to_ball3_13_Z@1 <-> to_rail_Z@50 [Mate]: SAR320-20_r:1 ↔ SAR3_ba:47
- to_ball3_13_YZ@1 <-> to_rail_YZ@50 [Angle] (0 deg): SAR320-20_r:1 ↔ SAR3_ba:47
- to_ball3_14_XY@1 <-> to_rail_XY@51 [Mate]: SAR320-20_r:1 ↔ SAR3_ba:48
- to_ball3_14_Z@1 <-> to_rail_Z@51 [Mate]: SAR320-20_r:1 ↔ SAR3_ba:48
- to_ball3_14_YZ@1 <-> to_rail_YZ@51 [Angle] (0 deg): SAR320-20_r:1 ↔ SAR3_ba:48
- to_ball3_15_XY@1 <-> to_rail_XY@52 [Mate]: SAR320-20_r:1 ↔ SAR3_ba:49
- to_ball3_15_Z@1 <-> to_rail_Z@52 [Mate]: SAR320-20_r:1 ↔ SAR3_ba:49
- to_ball3_15_YZ@1 <-> to_rail_YZ@52 [Angle] (0 deg): SAR320-20_r:1 ↔ SAR3_ba:49
- to_ball3_16_XY@1 <-> to_rail_XY@53 [Mate]: SAR320-20_r:1 ↔ SAR3_ba:50
- to_ball3_16_Z@1 <-> to_rail_Z@53 [Mate]: SAR320-20_r:1 ↔ SAR3_ba:50
- to_ball3_16_YZ@1 <-> to_rail_YZ@53 [Angle] (0 deg): SAR320-20_r:1 ↔ SAR3_ba:50
- to_ball3_17_XY@1 <-> to_rail_XY@54 [Mate]: SAR320-20_r:1 ↔ SAR3_ba:51
- to_ball3_17_Z@1 <-> to_rail_Z@54 [Mate]: SAR320-20_r:1 ↔ SAR3_ba:51
- to_ball3_17_YZ@1 <-> to_rail_YZ@54 [Angle] (0 deg): SAR320-20_r:1 ↔ SAR3_ba:51
- to_ball4_1_XY@1 <-> to_rail_XY@55 [Mate]: SAR320-20_r:1 ↔ SAR3_ba:52
- to_ball4_1_Z@1 <-> to_rail_Z@55 [Mate]: SAR320-20_r:1 ↔ SAR3_ba:52
- to_ball4_1_YZ@1 <-> to_rail_YZ@55 [Angle] (0 deg): SAR320-20_r:1 ↔ SAR3_ba:52
- to_ball4_2_XY@1 <-> to_rail_XY@56 [Mate]: SAR320-20_r:1 ↔ SAR3_ba:53
- to_ball4_2_Z@1 <-> to_rail_Z@56 [Mate]: SAR320-20_r:1 ↔ SAR3_ba:53
- to_ball4_2_YZ@1 <-> to_rail_YZ@56 [Angle] (0 deg): SAR320-20_r:1 ↔ SAR3_ba:53
- to_ball4_3_XY@1 <-> to_rail_XY@57 [Mate]: SAR320-20_r:1 ↔ SAR3_ba:54
- to_ball4_3_Z@1 <-> to_rail_Z@57 [Mate]: SAR320-20_r:1 ↔ SAR3_ba:54
- to_ball4_3_YZ@1 <-> to_rail_YZ@57 [Angle] (0 deg): SAR320-20_r:1 ↔ SAR3_ba:54
- to_ball4_4_XY@1 <-> to_rail_XY@58 [Mate]: SAR320-20_r:1 ↔ SAR3_ba:55
- to_ball4_4_Z@1 <-> to_rail_Z@58 [Mate]: SAR320-20_r:1 ↔ SAR3_ba:55
- to_ball4_4_YZ@1 <-> to_rail_YZ@58 [Angle] (0 deg): SAR320-20_r:1 ↔ SAR3_ba:55
- to_ball4_5_XY@1 <-> to_rail_XY@59 [Mate]: SAR320-20_r:1 ↔ SAR3_ba:56
- to_ball4_5_Z@1 <-> to_rail_Z@59 [Mate]: SAR320-20_r:1 ↔ SAR3_ba:56
- to_ball4_5_YZ@1 <-> to_rail_YZ@59 [Angle] (0 deg): SAR320-20_r:1 ↔ SAR3_ba:56
- to_ball4_6_XY@1 <-> to_rail_XY@60 [Mate]: SAR320-20_r:1 ↔ SAR3_ba:57
- to_ball4_6_Z@1 <-> to_rail_Z@60 [Mate]: SAR320-20_r:1 ↔ SAR3_ba:57
- to_ball4_6_YZ@1 <-> to_rail_YZ@60 [Angle] (0 deg): SAR320-20_r:1 ↔ SAR3_ba:57
- to_ball4_7_XY@1 <-> to_rail_XY@61 [Mate]: SAR320-20_r:1 ↔ SAR3_ba:58
- to_ball4_7_Z@1 <-> to_rail_Z@61 [Mate]: SAR320-20_r:1 ↔ SAR3_ba:58
- to_ball4_7_YZ@1 <-> to_rail_YZ@61 [Angle] (0 deg): SAR320-20_r:1 ↔ SAR3_ba:58
- to_ball4_8_XY@1 <-> to_rail_XY@62 [Mate]: SAR320-20_r:1 ↔ SAR3_ba:59
- to_ball4_8_Z@1 <-> to_rail_Z@62 [Mate]: SAR320-20_r:1 ↔ SAR3_ba:59
- to_ball4_8_YZ@1 <-> to_rail_YZ@62 [Angle] (0 deg): SAR320-20_r:1 ↔ SAR3_ba:59
- to_ball4_9_XY@1 <-> to_rail_XY@63 [Mate]: SAR320-20_r:1 ↔ SAR3_ba:60
- to_ball4_9_Z@1 <-> to_rail_Z@63 [Mate]: SAR320-20_r:1 ↔ SAR3_ba:60
- to_ball4_9_YZ@1 <-> to_rail_YZ@63 [Angle] (0 deg): SAR320-20_r:1 ↔ SAR3_ba:60
- to_ball4_10_XY@1 <-> to_rail_XY@64 [Mate]: SAR320-20_r:1 ↔ SAR3_ba:61
- to_ball4_10_Z@1 <-> to_rail_Z@64 [Mate]: SAR320-20_r:1 ↔ SAR3_ba:61
- to_ball4_10_YZ@1 <-> to_rail_YZ@64 [Angle] (0 deg): SAR320-20_r:1 ↔ SAR3_ba:61
- to_ball4_11_XY@1 <-> to_rail_XY@65 [Mate]: SAR320-20_r:1 ↔ SAR3_ba:62
- to_ball4_11_Z@1 <-> to_rail_Z@65 [Mate]: SAR320-20_r:1 ↔ SAR3_ba:62
- to_ball4_11_YZ@1 <-> to_rail_YZ@65 [Angle] (0 deg): SAR320-20_r:1 ↔ SAR3_ba:62
- to_ball4_12_XY@1 <-> to_rail_XY@66 [Mate]: SAR320-20_r:1 ↔ SAR3_ba:63
- to_ball4_12_Z@1 <-> to_rail_Z@66 [Mate]: SAR320-20_r:1 ↔ SAR3_ba:63
- to_ball4_12_YZ@1 <-> to_rail_YZ@66 [Angle] (0 deg): SAR320-20_r:1 ↔ SAR3_ba:63
- to_ball4_13_XY@1 <-> to_rail_XY@67 [Mate]: SAR320-20_r:1 ↔ SAR3_ba:64
- to_ball4_13_Z@1 <-> to_rail_Z@67 [Mate]: SAR320-20_r:1 ↔ SAR3_ba:64
- to_ball4_13_YZ@1 <-> to_rail_YZ@67 [Angle] (0 deg): SAR320-20_r:1 ↔ SAR3_ba:64
- to_ball4_14_XY@1 <-> to_rail_XY@68 [Mate]: SAR320-20_r:1 ↔ SAR3_ba:65
- to_ball4_14_Z@1 <-> to_rail_Z@68 [Mate]: SAR320-20_r:1 ↔ SAR3_ba:65
- to_ball4_14_YZ@1 <-> to_rail_YZ@68 [Angle] (0 deg): SAR320-20_r:1 ↔ SAR3_ba:65
- to_ball4_15_XY@1 <-> to_rail_XY@69 [Mate]: SAR320-20_r:1 ↔ SAR3_ba:66
- to_ball4_15_Z@1 <-> to_rail_Z@69 [Mate]: SAR320-20_r:1 ↔ SAR3_ba:66
- to_ball4_15_YZ@1 <-> to_rail_YZ@69 [Angle] (0 deg): SAR320-20_r:1 ↔ SAR3_ba:66
- to_ball4_16_XY@1 <-> to_rail_XY@70 [Mate]: SAR320-20_r:1 ↔ SAR3_ba:67
- to_ball4_16_Z@1 <-> to_rail_Z@70 [Mate]: SAR320-20_r:1 ↔ SAR3_ba:67
- to_ball4_16_YZ@1 <-> to_rail_YZ@70 [Angle] (0 deg): SAR320-20_r:1 ↔ SAR3_ba:67
- to_ball4_17_XY@1 <-> to_rail_XY@71 [Mate]: SAR320-20_r:1 ↔ SAR3_ba:68
- to_ball4_17_Z@1 <-> to_rail_Z@71 [Mate]: SAR320-20_r:1 ↔ SAR3_ba:68
- to_ball4_17_YZ@1 <-> to_rail_YZ@71 [Angle] (0 deg): SAR320-20_r:1 ↔ SAR3_ba:68
